# Autodesk Inventor assembly: Cool flippy boi
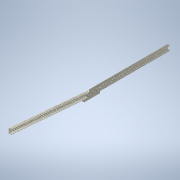
[picture p0: Inventor's stored thumbnail of the model, 180x180]
Saved by Autodesk Inventor 2020.1 (Build 241239000, 239)
## iProperties
Created: 2019-09-29
Part Number: Cool flippy boi
Document SubType Name: Assembly
Designer: 1069b
Author: 1069b
## Documents named in this file (4)
- C:\Users\1069b\Documents\Tower-Takeover-CAD\Parts\Cool flippy boi.iam
- C:\Users\1069b\Documents\Tower-Takeover-CAD\Parts\Structure\C-Channels\Aluminum\2-Wide\Aluminum C-Channel 1x2x1x35.ipt
- C:\Users\1069b\Documents\Tower-Takeover-CAD\Parts\Structure\C-Channels\Aluminum\2-Wide\Aluminum C-Channel 1x2x1x7.ipt
- C:\Users\1069b\Documents\Tower-Takeover-CAD\Parts\Structure\Standoffs & Couplers\Standoff 0.75''.ipt
## Components (6 placed, 3 different names)
1. Aluminum C-Channel 1x2x1x35:1 — Insert:1
2. Aluminum C-Channel 1x2x1x35:2 — Mate:1, Flush:1, Flush:2
3. Aluminum C-Channel 1x2x1x7:1 — Mate:1, Flush:1, Flush:2, Insert:1, Insert:2, Insert:3, Insert:4
4. Standoff 0.75'':1 — Insert:2
5. Standoff 0.75'':2 — Insert:4
6. Standoff 0.75'':3 — Insert:3
## Relationships (7: Insert 4, Flush 2, Mate 1)
- Mate:1: Aluminum C-Channel 1x2x1x35:2 ↔ Aluminum C-Channel 1x2x1x7:1
- Flush:1: Aluminum C-Channel 1x2x1x35:2 ↔ Aluminum C-Channel 1x2x1x7:1
- Flush:2: Aluminum C-Channel 1x2x1x35:2 ↔ Aluminum C-Channel 1x2x1x7:1
- Insert:1: Aluminum C-Channel 1x2x1x35:1 ↔ Aluminum C-Channel 1x2x1x7:1
- Insert:2: Aluminum C-Channel 1x2x1x7:1 ↔ Standoff 0.75'':1
- Insert:3: Aluminum C-Channel 1x2x1x7:1 ↔ Standoff 0.75'':3
- Insert:4: Aluminum C-Channel 1x2x1x7:1 ↔ Standoff 0.75'':2
